# Autodesk Inventor assembly: 팔각형 OV-PAM 5패턴
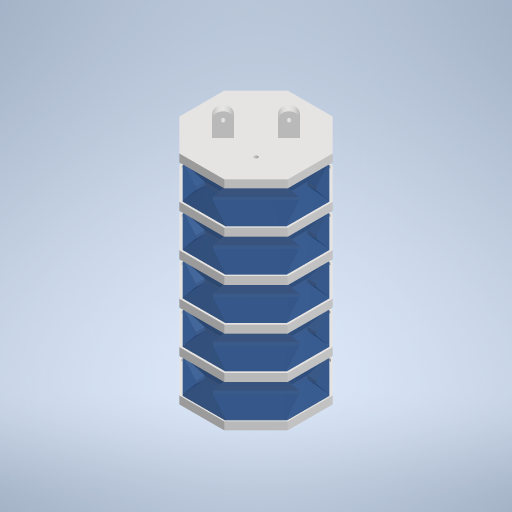
[picture p0: Inventor's stored thumbnail of the model, 512x512]
Saved by Autodesk Inventor 2024 (Build 280153000, 153)
## iProperties
Created: 2023-06-16
Part Number: 팔각형 OV-PAM 5패턴
Document SubType Name: Assembly
Designer: jsw
Author: jsw
## Documents named in this file (5)
- C:\승원\co-op\OV-PAM\OV-PAM_modeling\OV-PAM_5_patterns.iam
- C:\승원\co-op\OV-PAM\OV-PAM_modeling\OV-PAM_5_patterns_1f.ipt
- C:\승원\co-op\OV-PAM\OV-PAM_modeling\OV-PAM_top.ipt
- C:\승원\co-op\OV-PAM\OV-PAM_modeling\OV-PAM_bottom.ipt
- C:\승원\co-op\OV-PAM\OV-PAM_modeling\OV-PAM_ring.ipt
## Components (11 placed, 4 different names)
1. OV-PAM_top:1 — 메이트:1, 메이트:2, 메이트:3
2. OV-PAM_bottom:1 — 메이트:7, 메이트:8, 메이트:9
3. OV-PAM_5_patterns_1f:1 — 메이트:1, 메이트:2, 메이트:3, 메이트:4, 메이트:5, 메이트:6
4. OV-PAM_5_patterns_1f:2
5. OV-PAM_5_patterns_1f:3
6. OV-PAM_5_patterns_1f:4
7. OV-PAM_5_patterns_1f:5 — 메이트:7, 메이트:8, 메이트:9
8. OV-PAM_ring:1 — 메이트:4, 메이트:5, 메이트:6
9. OV-PAM_ring:2
10. OV-PAM_ring:3
11. OV-PAM_ring:4
## Component patterns: (5 elements, first: OV-PAM_5_patterns_1f:1), (4 elements, first: OV-PAM_ring:1)
## Relationships (9: Mate 9)
- 메이트:1 [Mate]: OV-PAM_top:1 ↔ OV-PAM_5_patterns_1f:1
- 메이트:2 [Mate]: OV-PAM_top:1 ↔ OV-PAM_5_patterns_1f:1
- 메이트:3 [Mate]: OV-PAM_top:1 ↔ OV-PAM_5_patterns_1f:1
- 메이트:4 [Mate]: OV-PAM_5_patterns_1f:1 ↔ OV-PAM_ring:1
- 메이트:5 [Mate]: OV-PAM_5_patterns_1f:1 ↔ OV-PAM_ring:1
- 메이트:6 [Mate]: OV-PAM_5_patterns_1f:1 ↔ OV-PAM_ring:1
- 메이트:7 [Mate]: OV-PAM_bottom:1 ↔ OV-PAM_5_patterns_1f:5
- 메이트:8 [Mate]: OV-PAM_bottom:1 ↔ OV-PAM_5_patterns_1f:5
- 메이트:9 [Mate]: OV-PAM_bottom:1 ↔ OV-PAM_5_patterns_1f:5
